# Autodesk Inventor assembly: AMR_Full_System_V1
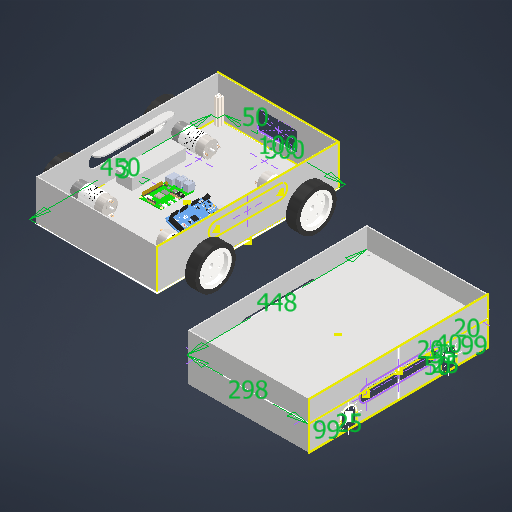
[picture p0: Inventor's stored thumbnail of the model, 512x512]
Saved by Autodesk Inventor 2026.2 (Build 302298010, 298A)
## iProperties
Created: 2026-03-25
Part Number: AMR_Full_System_V1
Document SubType Name: Assembly
Designer: Srishanth Dhondy
Author: Srishanth Dhondy
## Documents named in this file (10)
- D:\Cloud_Downloads\Srishanth\My Folder\Projects\AMR\CAD Design\AMR_Full_System_V1.iam
- D:\Cloud_Downloads\Srishanth\My Folder\Projects\AMR\CAD Design\AMR_Base_Box_V2.ipt
- D:\Cloud_Downloads\Srishanth\My Folder\Projects\AMR\CAD Design\AMR_Top_Basket.ipt
- D:\Cloud_Downloads\Srishanth\My Folder\Projects\AMR\CAD Design\Grab CAD\Wheels\Wheels v8\Wheels v8\Wheels v8.ipt
- D:\Cloud_Downloads\Srishanth\My Folder\Projects\AMR\CAD Design\Grab CAD\orange-planetary-gear-dc-motor-12v-970-rpm-14-5-n-cm-pg36m555-5-2k-1.snapshot.2\Motor\Motor\Motor.ipt
- D:\Cloud_Downloads\Srishanth\My Folder\Projects\AMR\CAD Design\Grab CAD\T-Slot\Aluminum Extrusion Bar\Aluminum Extrusion Bar\Aluminum Extrusion Bar.ipt
- D:\Cloud_Downloads\Srishanth\My Folder\Projects\AMR\CAD Design\Grab CAD\Arduino\Arduino Mega 2560 R3 v23\Arduino Mega 2560 R3 v23\Arduino Mega 2560 R3 v23.ipt
- D:\Cloud_Downloads\Srishanth\My Folder\Projects\AMR\CAD Design\Grab CAD\Raspberry Pi 4\Raspberry Pi 4 Model B\Raspberry Pi 4 Model B\Raspberry Pi 4 Model B.ipt
- D:\Cloud_Downloads\Srishanth\My Folder\Projects\AMR\CAD Design\AMR_Handle_Flap.ipt
- D:\Cloud_Downloads\Srishanth\My Folder\Projects\AMR\CAD Design\LiPo_Battery_Dummy.ipt
## Components (19 placed, 9 different names)
1. AMR_Base_Box_V2:1 — Rigid:1, Rigid:2, Rigid:3, Rigid:4, Rigid:5, Rigid:7, Rigid:8, Rigid:9, Rotational:2, Rotational:3
2. AMR_Top_Basket:1 — Rotational:1
3. Wheels v8:2 — Cylindrical:3
4. Wheels v8:3 — Cylindrical:4
5. Motor:1 — Rigid:8, Cylindrical:5
6. Motor:3 — Rigid:5, Cylindrical:4
7. Motor:4 — Rigid:7, Cylindrical:6
8. Aluminum Extrusion Bar:2 — Rigid:2
9. Aluminum Extrusion Bar:3 — Rigid:3
10. Aluminum Extrusion Bar:4 — Rigid:1, Rotational:1
11. Aluminum Extrusion Bar:5 — Rigid:4
12. Motor:5 — Rigid:9, Cylindrical:3
13. Wheels v8:5 — Cylindrical:5
14. Wheels v8:6 — Cylindrical:6
15. Arduino Mega 2560 R3 v23:1
16. Raspberry Pi 4 Model B:1
17. AMR_Handle_Flap:1 — Rotational:2
18. AMR_Handle_Flap:2 — Rotational:3
19. LiPo_Battery_Dummy:1
## Relationships (15: WeldJoint 8, CylindricalJoint 4, RevoluteJoint 3)
- Rigid:1 [WeldJoint]: AMR_Base_Box_V2:1 ↔ Aluminum Extrusion Bar:4
- Rigid:2 [WeldJoint]: AMR_Base_Box_V2:1 ↔ Aluminum Extrusion Bar:2
- Rigid:3 [WeldJoint]: AMR_Base_Box_V2:1 ↔ Aluminum Extrusion Bar:3
- Rigid:4 [WeldJoint]: AMR_Base_Box_V2:1 ↔ Aluminum Extrusion Bar:5
- Rigid:5 [WeldJoint]: AMR_Base_Box_V2:1 ↔ Motor:3
- Rigid:7 [WeldJoint]: AMR_Base_Box_V2:1 ↔ Motor:4
- Rigid:8 [WeldJoint]: AMR_Base_Box_V2:1 ↔ Motor:1
- Rigid:9 [WeldJoint]: AMR_Base_Box_V2:1 ↔ Motor:5
- Cylindrical:3: Wheels v8:2 ↔ Motor:5
- Cylindrical:4: Wheels v8:3 ↔ Motor:3
- Cylindrical:5: Motor:1 ↔ Wheels v8:5
- Cylindrical:6: Motor:4 ↔ Wheels v8:6
- Rotational:1 [RevoluteJoint] (8 mm): AMR_Top_Basket:1 ↔ Aluminum Extrusion Bar:4
- Rotational:2 [RevoluteJoint] (0.5 mm): AMR_Base_Box_V2:1 ↔ AMR_Handle_Flap:1
- Rotational:3 [RevoluteJoint] (0.5 mm): AMR_Base_Box_V2:1 ↔ AMR_Handle_Flap:2
